# Autodesk Inventor assembly: achterwiel
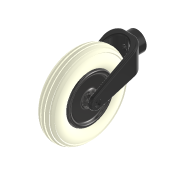
[picture p0: Inventor's stored thumbnail of the model, 180x180]
Saved by Autodesk Inventor 2020.3 (Build 243373000, 373)
## iProperties
Created: 2020-09-17
Part Number: achterwiel
Document SubType Name: Assembly
Designer: Svend
Author: Svend
## Documents named in this file (3)
- C:\Users\Svend\OneDrive\Documents\GitHub\Rolstoel\achterwiel.iam
- C:\Users\Svend\OneDrive\Documents\GitHub\Rolstoel\wielstuen.ipt
- C:\Users\Svend\OneDrive\Documents\GitHub\Rolstoel\achterwiel.ipt
## Components (2 placed, 2 different names)
1. wielstuen:1 — Mate:1, Mate:2
2. achterwiel:1 — Mate:1, Mate:2
## Relationships (2: Mate 2)
- Mate:1: wielstuen:1 ↔ achterwiel:1
- Mate:2: wielstuen:1 ↔ achterwiel:1
